# Autodesk Inventor assembly: BoardCutsTigerBurnHead2026
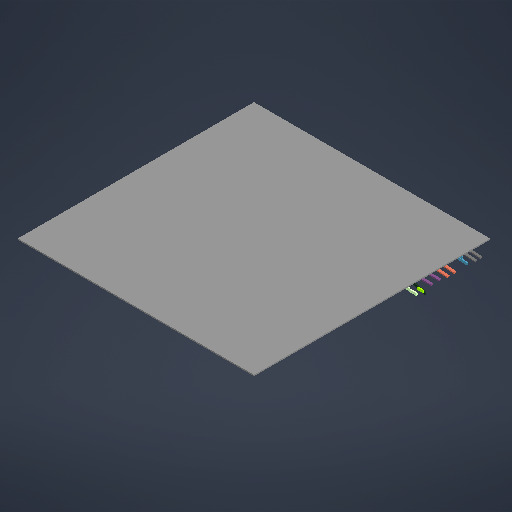
[picture p0: Inventor's stored thumbnail of the model, 512x512]
Saved by Autodesk Inventor 2027 (Build 310192000, 192)
## iProperties
Created: 2026-10-06
Part Number: BoardCutsTigerBurnHead2026
Document SubType Name: Assembly
Designer: lucas
Author: lucas
## Documents named in this file (33)
- C:\Users\lucas\OneDrive\Documents\Inventor\Tiger Burn Head Frame 2026\BoardCutsTigerBurnHead2026.iam
- C:\Users\lucas\OneDrive\Documents\Inventor\Tiger Burn Head Frame 2026\2x4x96.ipt
- C:\Users\lucas\OneDrive\Documents\Inventor\Tiger Burn Head Frame 2026\2x4x90.ipt
- C:\Users\lucas\OneDrive\Documents\Inventor\Tiger Burn Head Frame 2026\Base.ipt
- C:\Users\lucas\OneDrive\Documents\Inventor\Tiger Burn Head Frame 2026\Side piece.ipt
- C:\Users\lucas\OneDrive\Documents\Inventor\Tiger Burn Head Frame 2026\Rename.ipt
- C:\Users\lucas\OneDrive\Documents\Inventor\Tiger Burn Head Frame 2026\2x4x27.ipt
- C:\Users\lucas\OneDrive\Documents\Inventor\Tiger Burn Head Frame 2026\UpperEarDiagonalv2_MIR.ipt
- C:\Users\lucas\OneDrive\Documents\Inventor\Tiger Burn Head Frame 2026\Upper side diagonal.ipt
- C:\Users\lucas\OneDrive\Documents\Inventor\Tiger Burn Head Frame 2026\2x4x26.ipt
- C:\Users\lucas\OneDrive\Documents\Inventor\Tiger Burn Head Frame 2026\2x4x24.ipt
- C:\Users\lucas\OneDrive\Documents\Inventor\Tiger Burn Head Frame 2026\2x4x44.ipt
- C:\Users\lucas\OneDrive\Documents\Inventor\Tiger Burn Head Frame 2026\Top Diagonals.ipt
- C:\Users\lucas\OneDrive\Documents\Inventor\Tiger Burn Head Frame 2026\Renamev2_MIR.ipt
- C:\Users\lucas\OneDrive\Documents\Inventor\Tiger Burn Head Frame 2026\2x4x(24x43)_MIR.ipt
- C:\Users\lucas\OneDrive\Documents\Inventor\Tiger Burn Head Frame 2026\2x4x(Rename).ipt
- C:\Users\lucas\OneDrive\Documents\Inventor\Tiger Burn Head Frame 2026\2x4x88.ipt
- C:\Users\lucas\OneDrive\Documents\Inventor\Tiger Burn Head Frame 2026\Bottom jaw diagonals 2_MIR.ipt
- C:\Users\lucas\OneDrive\Documents\Inventor\Tiger Burn Head Frame 2026\2x4x30.ipt
- C:\Users\lucas\OneDrive\Documents\Inventor\Tiger Burn Head Frame 2026\SideConnectors.ipt
- C:\Users\lucas\OneDrive\Documents\Inventor\Tiger Burn Head Frame 2026\2x4x15.ipt
- C:\Users\lucas\OneDrive\Documents\Inventor\Tiger Burn Head Frame 2026\Upper side diagonal_MIR.ipt
- C:\Users\lucas\OneDrive\Documents\Inventor\Tiger Burn Head Frame 2026\2x4x13_MIR5.ipt
- C:\Users\lucas\OneDrive\Documents\Inventor\Tiger Burn Head Frame 2026\Top of head diagonals_MIR2.ipt
- C:\Users\lucas\OneDrive\Documents\Inventor\Tiger Burn Head Frame 2026\2x4x20.ipt
- C:\Users\lucas\OneDrive\Documents\Inventor\Tiger Burn Head Frame 2026\2x4x101.ipt
- C:\Users\lucas\OneDrive\Documents\Inventor\Tiger Burn Head Frame 2026\LowerEarDiagonals_MIR.ipt
- C:\Users\lucas\OneDrive\Documents\Inventor\Tiger Burn Head Frame 2026\Eyelids_MIR.ipt
- C:\Users\lucas\OneDrive\Documents\Inventor\Tiger Burn Head Frame 2026\2x4x39.ipt
- C:\Users\lucas\OneDrive\Documents\Inventor\Tiger Burn Head Frame 2026\2x4x38.ipt
- C:\Users\lucas\OneDrive\Documents\Inventor\Tiger Burn Head Frame 2026\2x4x24(with a cut)_MIR.ipt
- C:\Users\lucas\OneDrive\Documents\Inventor\Tiger Burn Head Frame 2026\2x4x13.ipt
- C:\Users\lucas\OneDrive\Documents\Inventor\Tiger Burn Head Frame 2026\2x4x(Rename)_MIR.ipt
## Components (112 placed, 32 different names)
1. Base:1 — Flush:3, Flush:4, Mate:1, Mate:2, Mate:3, Flush:5, Mate:4
2. 2x4x96:1 — Mate:1
3. 2x4x96:2
4. 2x4x96:3
5. 2x4x96:4
6. 2x4x92:1 — Mate:2
7. 2x4x92:2
8. Side piece:1 — Mate:3, Flush:5
9. Side piece:2
10. Side piece:3
11. Side piece:4
12. Side piece:5
13. Side piece:6
14. 2x4x34:1 — Mate:4
15. 2x4x34:2
16. 2x4x34:4
17. 2x4x34:5
18. 2x4x27:2
19. 2x4x27:3
20. UpperEarDiagonalv2_MIR:1
21. UpperEarDiagonalv2_MIR:2
22. Upper side diagonal:1
23. Upper side diagonal:2
24. 2x4x26:1
25. 2x4x26:2
26. 2x4x24:1
27. 2x4x24:2
28. 2x4x24:3
29. 2x4x24:4
30. 2x4x44:1
31. 2x4x44:2
32. Top Diagonals:1
33. Top Diagonals:2
34. Top Diagonals:3
35. Top Diagonals:4
36. Eyelidpt2_MIR:1
37. Eyelidpt2_MIR:2
38. 2x4x(24x43)_MIR:1
39. 2x4x11:1
40. 2x4x(24x43)_MIR:2
41. 2x4x(24x43)_MIR:3
42. 2x4x(24x43)_MIR:4
43. 2x4x26:3
44. 2x4x26:4
45. 2x4x26:5
46. 2x4x26:6
47. 2x4x88:1
48. 2x4x88:2
49. 2x4x88:3
50. 2x4x88:4
51. 2x4x88:5
52. 2x4x88:6
53. Bottom jaw diagonals 2_MIR:1
54. Bottom jaw diagonals 2_MIR:2
55. 2x4x30:1
56. 2x4x30:2
57. 2x4x88:7
58. 2x4x88:8
59. 2x4x88:9
60. 2x4x88:10
61. SideConnectors:1
62. SideConnectors:2
63. SideConnectors:3
64. SideConnectors:4
65. 2x4x15:1
66. 2x4x15:2
67. 2x4x15:3
68. 2x4x15:4
69. Upper side diagonal_MIR:1
70. Upper side diagonal_MIR:2
71. Upper side diagonal_MIR:3
72. Upper side diagonal_MIR:4
73. 2x4x13_MIR5:1
74. 2x4x13_MIR5:2
75. Top of head diagonals_MIR2:1
76. Top of head diagonals_MIR2:2
77. 2x4x20:1
78. 2x4x20:2
79. 2x4x20:3
80. 2x4x101:1
81. 2x4x101:2
82. 2x4x101:3
83. 2x4x101:4
84. 2x4x101:5
85. 2x4x101:6
86. 2x4x101:7
87. 2x4x101:8
88. LowerEarDiagonals_MIR:1
89. LowerEarDiagonals_MIR:2
90. Eyelids_MIR:1
91. Eyelids_MIR:2
92. 2x4x39:1
93. 2x4x39:2
94. 2x4x38:1
95. 2x4x38:2
96. 2x4x24:5
97. 2x4x24:6
98. 2x4x24(with a cut)_MIR:1
99. 2x4x24(with a cut)_MIR:2
100. 2x4x24(with a cut)_MIR:3
101. 2x4x24(with a cut)_MIR:4
102. 2x4x13:1
103. 2x4x13:2
104. 2x4x13:3
105. 2x4x13:4
106. 2x4x13:5
107. 2x4x13:6
108. 2x4x13:7
109. 2x4x13:8
110. 2x4x13:9
111. 2x4x13:10
112. 2x4x(Rename)_MIR:1
## Relationships (7: Mate 4, Flush 3)
- Flush:3: Base:1
- Flush:4: Base:1
- Mate:1: Base:1 ↔ 2x4x96:1
- Mate:2: Base:1 ↔ 2x4x92:1
- Mate:3: Base:1 ↔ Side piece:1
- Flush:5 (965.2 mm): Base:1 ↔ Side piece:1
- Mate:4: Base:1 ↔ 2x4x34:1
